# Autodesk Inventor assembly: Assembly1
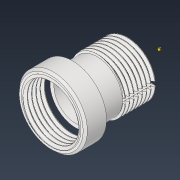
[picture p0: Inventor's stored thumbnail of the model, 180x180]
Saved by Autodesk Inventor 2022 (Build 260153000, 153)
## iProperties
Created: 2022-07-02
Part Number: Assembly1
Document SubType Name: Assembly
Designer: User
Author: User
## Documents named in this file (3)
- C:\Users\User\Desktop\test_twist_friction_lock\Assembly1.iam
- C:\Users\User\Desktop\test_twist_friction_lock\bottomPiece.ipt
- C:\Users\User\Desktop\test_twist_friction_lock\topPiece.ipt
## Components (2 placed, 2 different names)
1. bottomPiece:1 — Transitional:1, Angle:1, Mate:1
2. topPiece:1 — Transitional:1, Angle:1, Mate:1
## Relationships (3: Transitional 1, Angle 1, Mate 1)
- Transitional:1: bottomPiece:1 ↔ topPiece:1
- Angle:1 (0 deg): bottomPiece:1 ↔ topPiece:1
- Mate:1: bottomPiece:1 ↔ topPiece:1
